# Autodesk Inventor assembly: Vini-MyPnP
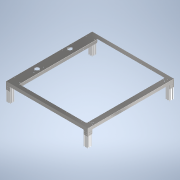
[picture p0: Inventor's stored thumbnail of the model, 180x180]
Saved by Autodesk Inventor 2020 (Build 240168000, 168)
## iProperties
Created: 2020-03-06
Part Number: Vini-MyPnP
Document SubType Name: Assembly
Designer: 10300812
Author: 10300812
## Documents named in this file (3)
- C:\Users\10300812\Documents\GitHub\MyPnP\Vini-MyPnP.iam
- C:\Users\10300812\Documents\GitHub\MyPnP\Gantry.ipt
- C:\Users\10300812\Documents\GitHub\MyPnP\User Library-8-AS-6-4040-VSLOT.ipt
## Components (5 placed, 2 different names)
1. Gantry:1 — Mate:1, Mate:2, Mate:3, Mate:4, Mate:5, Mate:6, Mate:7, Mate:8, Flush:4
2. User Library-8-AS-6-4040-VSLOT:1 — Mate:1, Mate:2, Flush:2, Flush:3, Flush:4
3. User Library-8-AS-6-4040-VSLOT:2 — Mate:3, Mate:4, Flush:3
4. User Library-8-AS-6-4040-VSLOT:3 — Mate:5, Mate:6, Flush:1
5. User Library-8-AS-6-4040-VSLOT:4 — Mate:7, Mate:8, Flush:1, Flush:2
## Relationships (12: Mate 8, Flush 4)
- Mate:1: Gantry:1 ↔ User Library-8-AS-6-4040-VSLOT:1
- Mate:2: Gantry:1 ↔ User Library-8-AS-6-4040-VSLOT:1
- Mate:3: Gantry:1 ↔ User Library-8-AS-6-4040-VSLOT:2
- Mate:4: Gantry:1 ↔ User Library-8-AS-6-4040-VSLOT:2
- Mate:5: Gantry:1 ↔ User Library-8-AS-6-4040-VSLOT:3
- Mate:6: Gantry:1 ↔ User Library-8-AS-6-4040-VSLOT:3
- Mate:7: Gantry:1 ↔ User Library-8-AS-6-4040-VSLOT:4
- Mate:8: Gantry:1 ↔ User Library-8-AS-6-4040-VSLOT:4
- Flush:1: User Library-8-AS-6-4040-VSLOT:3 ↔ User Library-8-AS-6-4040-VSLOT:4
- Flush:2: User Library-8-AS-6-4040-VSLOT:1 ↔ User Library-8-AS-6-4040-VSLOT:4
- Flush:3: User Library-8-AS-6-4040-VSLOT:1 ↔ User Library-8-AS-6-4040-VSLOT:2
- Flush:4 (-100 mm): Gantry:1 ↔ User Library-8-AS-6-4040-VSLOT:1
